# Autodesk Inventor assembly: Assembly4
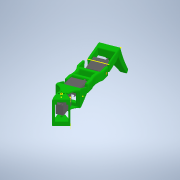
[picture p0: Inventor's stored thumbnail of the model, 180x180]
Saved by Autodesk Inventor 2022 (Build 260153000, 153)
## iProperties
Created: 2022-04-27
Part Number: Assembly4
Document SubType Name: Assembly
Designer: HP
Author: HP
## Documents named in this file (6)
- C:\Users\HP\Documents\Inventor\spider\Assembly4.iam
- C:\Users\HP\Documents\Inventor\spider\shoulder_link.ipt
- C:\Users\HP\Documents\Inventor\spider\Tower Pro MG996R_CPY.ipt
- C:\Users\HP\Documents\Inventor\spider\arm_link_up.ipt
- C:\Users\HP\Documents\Inventor\spider\arm_mid_link2.ipt
- C:\Users\HP\Documents\Inventor\spider\arm_under_link.ipt
## Components (7 placed, 5 different names)
1. shoulder_link:1 — Rotational:1
2. Tower Pro MG996R_CPY:1 — Rotational:1, Mate:1, Mate:2, Flush:1
3. arm_link_up:1 — Mate:1, Mate:2, Flush:1, Rotational:2
4. Tower Pro MG996R_CPY:2 — Rotational:2, Mate:3, Mate:4, Flush:2
5. arm_mid_link2:1 — Mate:3, Mate:4, Flush:2, Rotational:3
6. Tower Pro MG996R_CPY:3 — Mate:5, Mate:6, Flush:3, Rotational:3
7. arm_under_link:1 — Mate:5, Mate:6, Flush:3
## Relationships (12: Mate 6, RevoluteJoint 3, Flush 3)
- Rotational:1 [RevoluteJoint]: shoulder_link:1 ↔ Tower Pro MG996R_CPY:1
- Mate:1 (0.7112 mm): Tower Pro MG996R_CPY:1 ↔ arm_link_up:1
- Mate:2 (2.54 mm): Tower Pro MG996R_CPY:1 ↔ arm_link_up:1
- Flush:1 (19.05 mm): Tower Pro MG996R_CPY:1 ↔ arm_link_up:1
- Rotational:2 [RevoluteJoint] (-5.08 mm): arm_link_up:1 ↔ Tower Pro MG996R_CPY:2
- Mate:3: Tower Pro MG996R_CPY:2 ↔ arm_mid_link2:1
- Mate:4: Tower Pro MG996R_CPY:2 ↔ arm_mid_link2:1
- Flush:2 (-1.27 mm): Tower Pro MG996R_CPY:2 ↔ arm_mid_link2:1
- Mate:5 (17.78 mm): Tower Pro MG996R_CPY:3 ↔ arm_under_link:1
- Mate:6 (1.524 mm): Tower Pro MG996R_CPY:3 ↔ arm_under_link:1
- Flush:3 (4.191 mm): Tower Pro MG996R_CPY:3 ↔ arm_under_link:1
- Rotational:3 [RevoluteJoint]: arm_mid_link2:1 ↔ Tower Pro MG996R_CPY:3
